# Autodesk Inventor assembly: CSS2H-2512
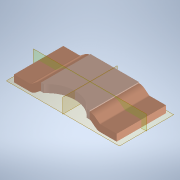
[picture p0: Inventor's stored thumbnail of the model, 180x180]
Saved by Autodesk Inventor 2020.1 (Build 241239000, 239)
## iProperties
Created: 2020-04-12
Part Number: CSS2H-2512
Document SubType Name: Assembly
Designer: yusaku
Author: yusaku
## Documents named in this file (3)
- C:\Users\Public\Documents\Altium\AD20\Library\libysk\3D Models\CSS2H-2512\CSS2H-2512.iam
- C:\Users\Public\Documents\Altium\AD20\Library\libysk\3D Models\CSS2H-2512\MANIFOLD_SOLID_BREP_547.ipt
- C:\Users\Public\Documents\Altium\AD20\Library\libysk\3D Models\CSS2H-2512\RESIST2512_3.ipt
## Components (3 placed, 2 different names)
1. MANIFOLD_SOLID_BREP_547:1 — Mate:2, Flush:1, Flush:2, Mate:3
2. RESIST2512_3:1 — Mate:1, Flush:1, Flush:2, Mate:3, Mate:5, Flush:3, Angle:1
3. MANIFOLD_SOLID_BREP_547:2 — Mate:4, Mate:5, Flush:3, Mate:6
## Relationships (10: Mate 6, Flush 3, Angle 1)
- Mate:1: RESIST2512_3:1
- Mate:2: MANIFOLD_SOLID_BREP_547:1
- Flush:1: MANIFOLD_SOLID_BREP_547:1 ↔ RESIST2512_3:1
- Flush:2: MANIFOLD_SOLID_BREP_547:1 ↔ RESIST2512_3:1
- Mate:3: MANIFOLD_SOLID_BREP_547:1 ↔ RESIST2512_3:1
- Mate:4: MANIFOLD_SOLID_BREP_547:2
- Mate:5: RESIST2512_3:1 ↔ MANIFOLD_SOLID_BREP_547:2
- Flush:3: RESIST2512_3:1 ↔ MANIFOLD_SOLID_BREP_547:2
- Angle:1 (0 deg): RESIST2512_3:1
- Mate:6 (-1.525 mm): MANIFOLD_SOLID_BREP_547:2
